# Autodesk Inventor assembly: HUB BOTTOM
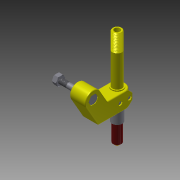
[picture p0: Inventor's stored thumbnail of the model, 180x180]
Saved by Autodesk Inventor 2013 (Build 170138000, 138)
## iProperties
Created: 2013-11-26
Part Number: HUB BOTTOM
Document SubType Name: Assembly
Designer: employee
Author: employee
## Documents named in this file (8)
- C:\Users\employee\Desktop\GUS Simpson\HUB BOTTOM.iam
- C:\Users\employee\Desktop\GUS Simpson\HUB BOTTOM.ipt
- C:\Users\employee\Desktop\GUS Simpson\M8x55.ipt
- C:\Users\employee\Desktop\GUS Simpson\M8 WASHER.ipt
- C:\Users\employee\Desktop\GUS Simpson\M8 NUT.ipt
- C:\Users\employee\Desktop\GUS Simpson\M3x20.ipt
- C:\Users\employee\Desktop\GUS Simpson\M3 NUT.ipt
- C:\Users\employee\Desktop\GUS Simpson\_UBIS.ipt
## Components (9 placed, 7 different names)
1. HUB BOTTOM:1 — Insert:1, Angle:1, Insert:2, Insert:4, Insert:5, Insert:6, Angle:2, Insert:7, Angle:3, Insert:8
2. M8x55:1 — Insert:1, Angle:1
3. M8 WASHER:1 — Insert:2, Insert:3
4. M8 NUT:1 — Insert:3
5. M3x20:1 — Insert:5
6. M3x20:2 — Insert:4
7. M3 NUT:1 — Insert:6, Angle:2
8. M3 NUT:2 — Insert:7, Angle:3
9. _UBIS:1 — Insert:8
## Relationships (11: Insert 8, Angle 3)
- Insert:1: HUB BOTTOM:1 ↔ M8x55:1
- Angle:1 (0 deg): HUB BOTTOM:1 ↔ M8x55:1
- Insert:2: HUB BOTTOM:1 ↔ M8 WASHER:1
- Insert:3 (25 mm): M8 WASHER:1 ↔ M8 NUT:1
- Insert:4: HUB BOTTOM:1 ↔ M3x20:2
- Insert:5: HUB BOTTOM:1 ↔ M3x20:1
- Insert:6: HUB BOTTOM:1 ↔ M3 NUT:1
- Angle:2 (0 deg): HUB BOTTOM:1 ↔ M3 NUT:1
- Insert:7: HUB BOTTOM:1 ↔ M3 NUT:2
- Angle:3 (0 deg): HUB BOTTOM:1 ↔ M3 NUT:2
- Insert:8: HUB BOTTOM:1 ↔ _UBIS:1
